# Autodesk Inventor assembly: Door-Assembly-Group2
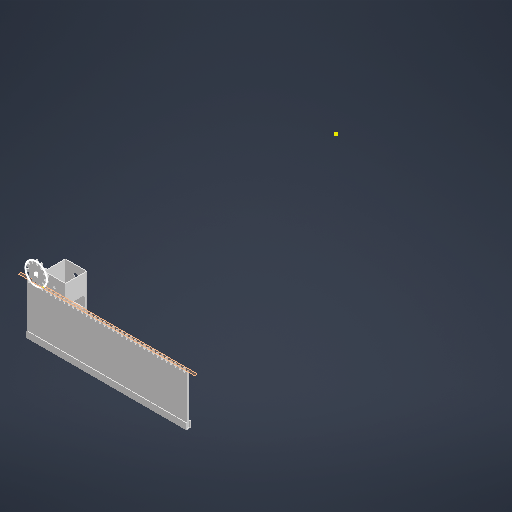
[picture p0: Inventor's stored thumbnail of the model, 512x512]
Saved by Autodesk Inventor 2026.1 (Build 301233000, 233)
## iProperties
Created: 2026-02-27
Part Number: Door-Assembly-Group2
Document SubType Name: Assembly
Designer: ba2032
Author: ba2032
## Documents named in this file (5)
- C:\Users\ba2032\Documents\Door-Assembly-Group2.iam
- H:\CAD Project\DoorPinion.ipt
- H:\CAD Project\Door.ipt
- H:\CAD Project\DoorRail.ipt
- H:\CAD Project\MotorHolder.ipt
## Components (4 placed, 4 different names)
1. DoorPinion:1 — Mate:1, Flush:1, Flush:2
2. Door:1 — Flush:2, Flush:3, Slider:1
3. DoorRail:1 — Flush:4, Slider:1, Mate:2
4. MotorHolder:1
## Relationships (7: Flush 4, Mate 2, TranslationJoint 1)
- Mate:1: DoorPinion:1
- Flush:1: DoorPinion:1
- Flush:2: DoorPinion:1 ↔ Door:1
- Flush:3 (10.043 mm): Door:1
- Flush:4 (-1 mm): DoorRail:1
- Slider:1 [TranslationJoint]: Door:1 ↔ DoorRail:1
- Mate:2 (-10 mm): DoorRail:1
